# Autodesk Inventor assembly: DriveMotorAssem_MIR
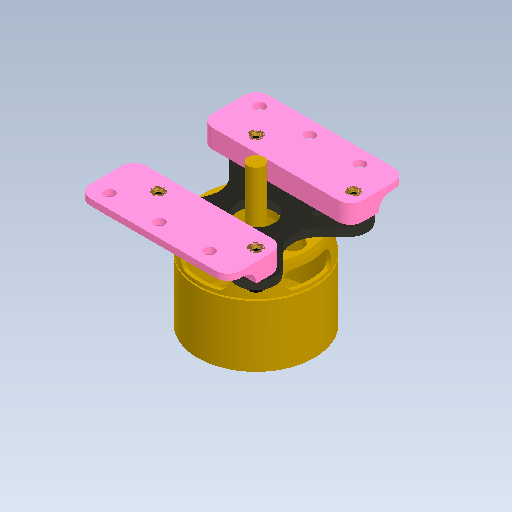
[picture p0: Inventor's stored thumbnail of the model, 512x512]
Saved by Autodesk Inventor 2023 (Build 270158000, 158)
## iProperties
Created: 2023-03-30
Part Number: DriveMotorAssem_MIR
Document SubType Name: Assembly
Designer: Dave
Mass: 268.152 g
Surface Area: 522.44 cm^2
Volume: 82.9291 cm^3
Density: 3.2335 g/cm^3
Author: Dave
## Documents named in this file (7)
- C:\Users\Dave\Documents\GitHub\BehrendURCMechanical\CAD\Chassis V3\DriveMotorAssem\DriveMotorAssem_MIR.iam
- C:\Users\Dave\Documents\GitHub\BehrendURCMechanical\CAD\Chassis V3\DriveMotorPlate_MIR.ipt
- C:\Users\Dave\Documents\GitHub\BehrendURCMechanical\CAD\Chassis V3\DriveMotorAssem\Drive Motor_MIR.ipt
- C:\Users\Dave\Downloads\91290A148_Alloy Steel Socket Head Screw_MIR.ipt
- C:\Users\Dave\Downloads\94180A351_Tapered Heat-Set Inserts for Plastic_MIR.ipt
- C:\Users\Dave\Documents\GitHub\BehrendURCMechanical\CAD\Chassis V3\DriveMotorAssem\DriveMotorMount5_MIR2.ipt
- C:\Users\Dave\Documents\GitHub\BehrendURCMechanical\CAD\Chassis V3\DriveMotorAssem\DriveMotorMount5_MIR1_MIR.ipt
## Components (12 placed, 6 different names)
1. DriveMotorPlate_MIR:1 — Insert:2, Insert:1, Insert:9, Insert:10, Insert:11, Insert:12, Insert:13, Insert:18, Insert:17
2. Drive Motor_MIR:1 — Insert:2, Insert:1
3. 91290A148_Alloy Steel Socket Head Screw_MIR:1 — Insert:9
4. 94180A351_Tapered Heat-Set Inserts for Plastic_MIR:1 — Insert:20
5. 91290A148_Alloy Steel Socket Head Screw_MIR:2 — Insert:10, Mate:1
6. 94180A351_Tapered Heat-Set Inserts for Plastic_MIR:2 — Insert:19
7. 91290A148_Alloy Steel Socket Head Screw_MIR:3 — Insert:11
8. 94180A351_Tapered Heat-Set Inserts for Plastic_MIR:3 — Insert:16
9. 91290A148_Alloy Steel Socket Head Screw_MIR:4 — Insert:12
10. 94180A351_Tapered Heat-Set Inserts for Plastic_MIR:4 — Insert:15
11. DriveMotorMount5_MIR2:1 — Insert:16, Insert:15, Mate:1, Insert:13
12. DriveMotorMount5_MIR1_MIR:1 — Insert:20, Insert:19, Insert:18, Insert:17
## Relationships (14: Insert 13, Mate 1)
- Insert:2: DriveMotorPlate_MIR:1 ↔ Drive Motor_MIR:1
- Insert:1: DriveMotorPlate_MIR:1 ↔ Drive Motor_MIR:1
- Insert:9: DriveMotorPlate_MIR:1 ↔ 91290A148_Alloy Steel Socket Head Screw_MIR:1
- Insert:10: DriveMotorPlate_MIR:1 ↔ 91290A148_Alloy Steel Socket Head Screw_MIR:2
- Insert:11: DriveMotorPlate_MIR:1 ↔ 91290A148_Alloy Steel Socket Head Screw_MIR:3
- Insert:12: DriveMotorPlate_MIR:1 ↔ 91290A148_Alloy Steel Socket Head Screw_MIR:4
- Insert:16: 94180A351_Tapered Heat-Set Inserts for Plastic_MIR:3 ↔ DriveMotorMount5_MIR2:1
- Insert:15: 94180A351_Tapered Heat-Set Inserts for Plastic_MIR:4 ↔ DriveMotorMount5_MIR2:1
- Mate:1: 91290A148_Alloy Steel Socket Head Screw_MIR:2 ↔ DriveMotorMount5_MIR2:1
- Insert:13: DriveMotorPlate_MIR:1 ↔ DriveMotorMount5_MIR2:1
- Insert:20: 94180A351_Tapered Heat-Set Inserts for Plastic_MIR:1 ↔ DriveMotorMount5_MIR1_MIR:1
- Insert:19: 94180A351_Tapered Heat-Set Inserts for Plastic_MIR:2 ↔ DriveMotorMount5_MIR1_MIR:1
- Insert:18: DriveMotorPlate_MIR:1 ↔ DriveMotorMount5_MIR1_MIR:1
- Insert:17: DriveMotorPlate_MIR:1 ↔ DriveMotorMount5_MIR1_MIR:1
